# Autodesk Inventor assembly: webots_Ldownframe
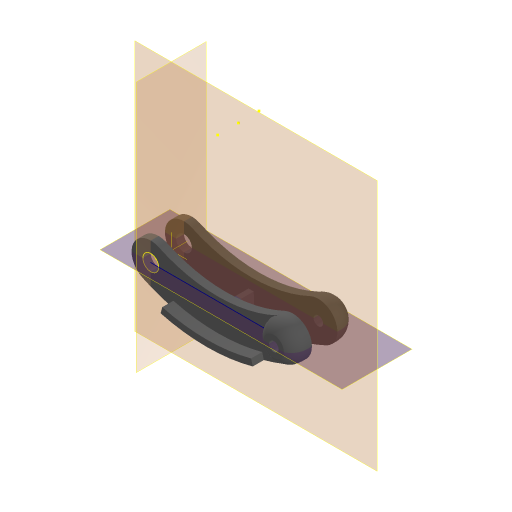
[picture p0: Inventor's stored thumbnail of the model, 512x512]
Saved by Autodesk Inventor 2023 (Build 270158000, 158)
## iProperties
Created: 2022-06-23
Part Number: webots_Ldownframe
Document SubType Name: Assembly
Designer: BioRoLaT470S
Mass: 32 g
Surface Area: 170.529 cm^2
Volume: 36.1072 cm^3
Density: 0.88625 g/cm^3
Author: BioRoLaT470S
## Documents named in this file (2)
- C:\Users\guanlunlu\Desktop\MBD_CORGI\CAD\webots_Ldownframe.iam
- C:\Users\guanlunlu\Desktop\MBD_CORGI\R100_properties\組合檔_v4\下框2.ipt
## Components (1 placed, 1 different names)
1. 下框2:1 — Mate:1, Mate:2, Flush:1
## Relationships (3: Mate 2, Flush 1)
- Mate:1: 下框2:1
- Mate:2: 下框2:1
- Flush:1: 下框2:1
